# Autodesk Inventor assembly: BoxWithCover
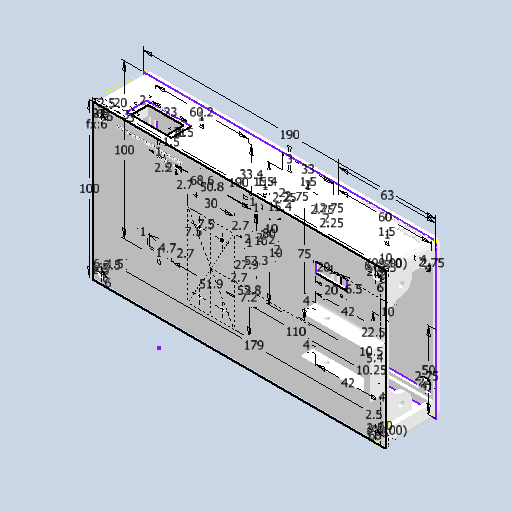
[picture p0: Inventor's stored thumbnail of the model, 512x512]
Saved by Autodesk Inventor 2023 (Build 270158000, 158)
## iProperties
Created: 2022-10-22
Part Number: BoxWithCover
Document SubType Name: Assembly
Designer: Miner
Author: Miner
## Documents named in this file (3)
- D:\AKFS\OneDrive - RMIT University\0. Main Research\139. Spectral Camera\01 GitHub\3D Design and Parts\Enclosure with Cover.iam
- D:\AKFS\OneDrive - RMIT University\0. Main Research\139. Spectral Camera\01 GitHub\3D Design and Parts\Source files\Part10 Enclosure.ipt
- D:\AKFS\OneDrive - RMIT University\0. Main Research\139. Spectral Camera\01 GitHub\3D Design and Parts\Source files\Part09 Enclosure cover.ipt
## Components (2 placed, 2 different names)
1. Part10 Enclosure:1 — Rotational:1
2. Part09 Enclosure cover:1 — Rotational:1
## Relationships (1: RevoluteJoint 1)
- Rotational:1 [RevoluteJoint]: Part10 Enclosure:1 ↔ Part09 Enclosure cover:1
